# Autodesk Inventor assembly: ptn60_uni_1_asm
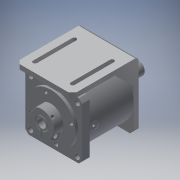
[picture p0: Inventor's stored thumbnail of the model, 180x180]
Saved by Autodesk Inventor 2018 (Build 220112000, 112)
## iProperties
Created: 2005-10-28
Part Number: ptn60_uni_1_asm
Document SubType Name: Assembly
Designer: m234547
Sending System: PRO/ENGINEER BY PARAMETRIC TECHNOLOGY CORPORATION, 2005170
Preprocessor: PRO/ENGINEER BY PARAMETRIC TECHNOLOGY CORPORATION, 2005170
Title: PLE60_UNI_1_ASM
Author: Ille
Revision Number: 7LAST_VERSION
## Documents named in this file (5)
- E:\step motor\NEMA23\ptn60_uni_1_asm.iam
- E:\step motor\NEMA23\PLE60_UNI_1.ipt
- E:\step motor\NEMA23\210-240_065_002.ipt
- E:\step motor\NEMA23\M4_10.ipt
- E:\step motor\mount.ipt
## Components (4 placed, 4 different names)
1. PLE60_UNI_1_0 — Mate:1, Mate:2, Mate:3
2. 210-240_065_002_1
3. M4_10_2
4. mount:1 — Mate:1, Mate:2, Mate:3
## Relationships (3: Mate 3)
- Mate:1: PLE60_UNI_1_0 ↔ mount:1
- Mate:2: PLE60_UNI_1_0 ↔ mount:1
- Mate:3: PLE60_UNI_1_0 ↔ mount:1
